# Autodesk Inventor assembly: ODrive Pack
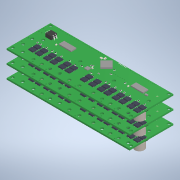
[picture p0: Inventor's stored thumbnail of the model, 180x180]
Saved by Autodesk Inventor 2022.2 (Build 262287000, 287)
## iProperties
Created: 2022-01-17
Part Number: ODrive Pack
Document SubType Name: Assembly
Designer: Jochen
Author: Jochen
## Documents named in this file (2)
- D:\Projects\Chewbacca\CAD\Common\odrive\ODrive Pack.iam
- D:\Projects\Chewbacca\CAD\Common\odrive\ODrive 3.5.iam
## Components (3 placed, 1 different names)
1. ODrive 3.5:1 [sub-assembly] — Mate:1, Flush:1, Mate:3
2. ODrive 3.5:2 [sub-assembly] — Flush:1, Flush:2, Mate:2, Mate:4
3. ODrive 3.5:3 [sub-assembly] — Mate:1, Flush:2, Mate:2, Mate:3, Mate:4
## Relationships (6: Mate 4, Flush 2)
- Mate:1 (13 mm): ODrive 3.5:1 ↔ ODrive 3.5:3
- Flush:1: ODrive 3.5:1 ↔ ODrive 3.5:2
- Flush:2: ODrive 3.5:2 ↔ ODrive 3.5:3
- Mate:2 (13 mm): ODrive 3.5:2 ↔ ODrive 3.5:3
- Mate:3: ODrive 3.5:1 ↔ ODrive 3.5:3
- Mate:4: ODrive 3.5:2 ↔ ODrive 3.5:3
